# Autodesk Inventor assembly: deflector
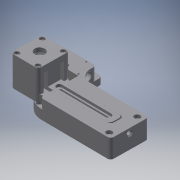
[picture p0: Inventor's stored thumbnail of the model, 180x180]
Saved by Autodesk Inventor 2019.3 (Build 233278000, 278)
## iProperties
Created: 2020-08-24
Part Number: deflector
Material: Generisch
Document SubType Name: Assembly
Designer: Nicolas Frick
Author: Nicolas Frick
## Documents named in this file (6)
- C:\Users\Nicolas Frick\Sync\OneDrive\airhockeybot\mechanical_design\inventor\deflector.iam
- C:\Users\Nicolas Frick\Sync\OneDrive\airhockeybot\mechanical_design\inventor\Bearing_support_outside.ipt
- C:\Users\Nicolas Frick\Sync\OneDrive\airhockeybot\mechanical_design\inventor\Bearing_support_inside.ipt
- C:\Users\Nicolas Frick\Sync\OneDrive\airhockeybot\mechanical_design\inventor\Fixture_mid.ipt
- C:\Users\Nicolas Frick\Sync\OneDrive\airhockeybot\mechanical_design\inventor\Fixture_linear_mid.ipt
- C:\Users\Nicolas Frick\Sync\OneDrive\airhockeybot\mechanical_design\inventor\Pulley.iam
## Components (5 placed, 5 different names)
1. Bearing_support_outside:1 — Passend:15, Fluchtend:1, Fluchtend:2
2. Bearing_support_inside:1 — Passend:15, Fluchtend:1, Fluchtend:2, Fluchtend:3, Passend:19, Passend:20, Passend:26
3. Fixture_mid:1 — Fluchtend:3, Passend:19, Passend:20, Passend:21, Fluchtend:4, Passend:25
4. Fixture_linear_mid:1 — Passend:21, Fluchtend:4, Passend:25
5. Pulley:1 [sub-assembly] — Passend:26
## Relationships (10: Mate 6, Flush 4)
- Passend:15 [Mate]: Bearing_support_outside:1 ↔ Bearing_support_inside:1
- Fluchtend:1 [Flush]: Bearing_support_outside:1 ↔ Bearing_support_inside:1
- Fluchtend:2 [Flush]: Bearing_support_outside:1 ↔ Bearing_support_inside:1
- Fluchtend:3 [Flush] (-25 mm): Bearing_support_inside:1 ↔ Fixture_mid:1
- Passend:19 [Mate]: Bearing_support_inside:1 ↔ Fixture_mid:1
- Passend:20 [Mate] (4.996 mm): Bearing_support_inside:1 ↔ Fixture_mid:1
- Passend:21 [Mate]: Fixture_mid:1 ↔ Fixture_linear_mid:1
- Fluchtend:4 [Flush]: Fixture_mid:1 ↔ Fixture_linear_mid:1
- Passend:25 [Mate]: Fixture_mid:1 ↔ Fixture_linear_mid:1
- Passend:26 [Mate]: Bearing_support_inside:1 ↔ Pulley:1
